# Autodesk Inventor assembly: PIP-KL, spolrotor_03 [2020-11-22]
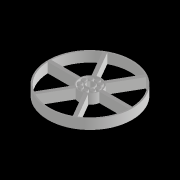
[picture p0: Inventor's stored thumbnail of the model, 180x180]
Saved by Autodesk Inventor 2020 (Build 240168000, 168)
## iProperties
Created: 2020-11-22
Part Number: PIP-KL, spolrotor_03 [2020-11-22]
Document SubType Name: Assembly
Designer: Gottfrid
Author: Gottfrid
## Documents named in this file (3)
- D:\PROJEKT\GENERATOR V.1\3D-filer [2020-11-21]\03\PIP-KL, spolrotor_03 [2020-11-22].iam
- D:\PROJEKT\GENERATOR V.1\3D-filer [2020-11-21]\03\PIP-KL_parametriserad_03 [2020-11-22].ipt
- D:\PROJEKT\GENERATOR V.1\3D-filer [2020-11-21]\03\Spol_rotor_parameteriserad_03 [2020-11-22].ipt
## Components (2 placed, 2 different names)
1. PIP-KL_parametriserad_03 [2020-11-22]:1 — Rigid:2
2. Spol_rotor_parameteriserad_03 [2020-11-22]:1 — Rigid:2
## Relationships (1: WeldJoint 1)
- Rigid:2 [WeldJoint]: PIP-KL_parametriserad_03 [2020-11-22]:1 ↔ Spol_rotor_parameteriserad_03 [2020-11-22]:1
